# Autodesk Inventor assembly: Ensamblaje_Engranes
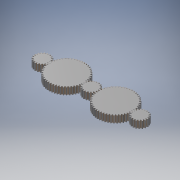
[picture p0: Inventor's stored thumbnail of the model, 180x180]
Saved by Autodesk Inventor 2018 (Build 220112000, 112)
## iProperties
Created: 2021-01-30
Part Number: Ensamblaje_Engranes
Material: Genérico
Document SubType Name: Assembly
Designer: rotje
Author: rotje
## Documents named in this file (3)
- C:\Users\rotje\Documents\Inventor\MSF\Ensamblaje_Engranes.iam
- C:\Users\rotje\Documents\Inventor\MSF\Ensamblaje_Engranes\Design Accelerator\Engranajes rectos1.iam
- C:\Users\rotje\Documents\Inventor\MSF\Ensamblaje_Engranes\Design Accelerator\Engranajes rectos2.iam
## Components (5 placed, 1 different names)
1. Engranajes rectos:1 [sub-assembly] — Coincidencia:1, Coincidencia:2, Nivelación:1, Tangente:1, Rotación:1
2. Engranajes rectos:2 [sub-assembly] — Nivelación:1, Tangente:1, Coincidencia:3, Tangente:2, Rotación:1, Rotación:2
3. Engranajes rectos:3 [sub-assembly] — Tangente:2, Coincidencia:4, Coincidencia:5, Tangente:3, Rotación:2, Rotación:3
4. Engranajes rectos:4 [sub-assembly] — Coincidencia:6, Tangente:3, Tangente:4, Coincidencia:8, Rotación:3, Rotación:4
5. Engranajes rectos:5 [sub-assembly] — Coincidencia:7, Tangente:4, Coincidencia:9, Rotación:4
## Relationships (18: Mate 9, Tangent 4, RelateRotation 4, Flush 1)
- Coincidencia:1 [Mate]: Engranajes rectos:1
- Coincidencia:2 [Mate]: Engranajes rectos:1
- Nivelación:1 [Flush]: Engranajes rectos:1 ↔ Engranajes rectos:2
- Tangente:1: Engranajes rectos:1 ↔ Engranajes rectos:2
- Coincidencia:3 [Mate]: Engranajes rectos:2
- Tangente:2: Engranajes rectos:2 ↔ Engranajes rectos:3
- Coincidencia:4 [Mate]: Engranajes rectos:3
- Coincidencia:5 [Mate]: Engranajes rectos:3
- Coincidencia:6 [Mate]: Engranajes rectos:4
- Coincidencia:7 [Mate]: Engranajes rectos:5
- Tangente:3: Engranajes rectos:3 ↔ Engranajes rectos:4
- Tangente:4: Engranajes rectos:4 ↔ Engranajes rectos:5
- Coincidencia:8 [Mate]: Engranajes rectos:4
- Coincidencia:9 [Mate]: Engranajes rectos:5
- Rotación:1 [RelateRotation] (0.4 ul): Engranajes rectos:1 ↔ Engranajes rectos:2
- Rotación:2 [RelateRotation] (2.5 ul): Engranajes rectos:2 ↔ Engranajes rectos:3
- Rotación:3 [RelateRotation] (0.4 ul): Engranajes rectos:3 ↔ Engranajes rectos:4
- Rotación:4 [RelateRotation] (2.5 ul): Engranajes rectos:4 ↔ Engranajes rectos:5
